# Autodesk Inventor assembly: Сборка3
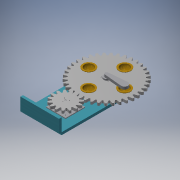
[picture p0: Inventor's stored thumbnail of the model, 180x180]
Saved by Autodesk Inventor 2018.3 (Build 223284000, 284)
## iProperties
Created: 2018-06-07
Part Number: Сборка3
Material: Типовые
Document SubType Name: Assembly
Designer: Leancher
Author: Leancher
## Documents named in this file (10)
- C:\Users\Leancher\GoogleDrive\My_project\Механика\Кофемашина\Inventor\Сборка.iam
- C:\Users\Leancher\GoogleDrive\My_project\Механика\Кофемашина\Inventor\Основание.ipt
- C:\Users\Leancher\GoogleDrive\My_project\Механика\Кофемашина\Inventor\Фильтр.ipt
- C:\Users\Leancher\GoogleDrive\My_project\Механика\Кофемашина\Inventor\Деталь1.ipt
- C:\Users\Leancher\GoogleDrive\My_project\Механика\Кофемашина\Inventor\Фланец.ipt
- C:\Users\Leancher\GoogleDrive\My_project\Механика\Кофемашина\Inventor\Зубчатая передача1.iam
- C:\Users\Leancher\GoogleDrive\My_project\Механика\Кофемашина\Inventor\Ось.ipt
- C:\Users\Leancher\GoogleDrive\My_project\Механика\Кофемашина\Inventor\MotorNema14.ipt
- C:\Users\Leancher\GoogleDrive\My_project\Механика\Кофемашина\Inventor\Проставка шестерни.ipt
- C:\Users\Leancher\GoogleDrive\My_project\Механика\Кофемашина\Inventor\Держатель двигателя.ipt
## Components (12 placed, 9 different names)
1. Основание:1 — Вставка:1, Заподлицо:3, Заподлицо:4
2. Лейка — Совмещение:3
3. Зубчатая передача:1 [sub-assembly] — Совмещение:5, Вставка:3, Совмещение:6, Совмещение:7
4. Фланец:1 — Совмещение:5, Вставка:3, Совмещение:6
5. Ось:1 — Вставка:1, Совмещение:3, Заподлицо:1, Заподлицо:2
6. MotorNema14:1 — Вставка:2
7. Проставка шестерни:1 — Заподлицо:1, Заподлицо:2, Совмещение:7
8. Держатель двигателя:1 — Заподлицо:3, Заподлицо:4, Вставка:2
9. Фильтр:1
10. Фильтр:2
11. Фильтр:3
12. Фильтр:4
## Component patterns: (4 elements, first: Фильтр:1)
## Relationships (11: Mate 4, Flush 4, Insert 3)
- Вставка:1 [Insert]: Основание:1 ↔ Ось:1
- Совмещение:3 [Mate]: Лейка ↔ Ось:1
- Заподлицо:1 [Flush]: Ось:1 ↔ Проставка шестерни:1
- Заподлицо:2 [Flush]: Ось:1 ↔ Проставка шестерни:1
- Заподлицо:3 [Flush]: Основание:1 ↔ Держатель двигателя:1
- Заподлицо:4 [Flush]: Основание:1 ↔ Держатель двигателя:1
- Вставка:2 [Insert]: MotorNema14:1 ↔ Держатель двигателя:1
- Совмещение:5 [Mate]: Зубчатая передача:1 ↔ Фланец:1
- Вставка:3 [Insert]: Зубчатая передача:1 ↔ Фланец:1
- Совмещение:6 [Mate]: Зубчатая передача:1 ↔ Фланец:1
- Совмещение:7 [Mate]: Зубчатая передача:1 ↔ Проставка шестерни:1
